# Autodesk Inventor assembly: fight_robot_fin1
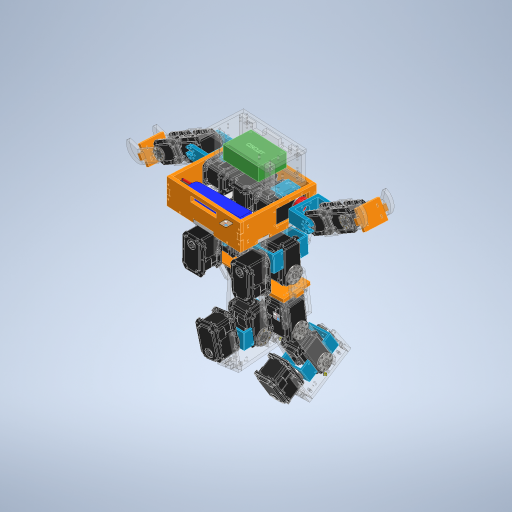
[picture p0: Inventor's stored thumbnail of the model, 512x512]
Saved by Autodesk Inventor 2024 (Build 280153000, 153)
## iProperties
Created: 2024-09-14
Part Number: fight_robot_fin1
Document SubType Name: Assembly
Designer: jmha0
Author: jmha0
## Documents named in this file (16)
- C:\Users\jmha0\OneDrive\바탕 화면\19th_intern_hjm_fight_robot\fight_robot_fin1.iam
- C:\Users\jmha0\OneDrive\바탕 화면\19th_intern_hjm_fight_robot\Lower_Body\waist\waist_fin1.iam
- C:\Users\jmha0\OneDrive\바탕 화면\19th_intern_hjm_fight_robot\Lower_Body\pelvis_w_motor\pelvis_w_motor_fin1.iam
- C:\Users\jmha0\OneDrive\바탕 화면\19th_intern_hjm_fight_robot\Lower_Body\pelvis_w_motor\pelvis_w_motor_fin1_opp.iam
- C:\Users\jmha0\OneDrive\바탕 화면\19th_intern_hjm_fight_robot\Lower_Body\knee_w_motor\knee_w_motor_fin1.iam
- C:\Users\jmha0\OneDrive\바탕 화면\19th_intern_hjm_fight_robot\Lower_Body\ankle_w_motor\ankle_w_motor_fin1.iam
- C:\Users\jmha0\OneDrive\바탕 화면\19th_intern_hjm_fight_robot\Lower_Body\ankle_w_motor\ankle_w_motor_fin1_opp.iam
- C:\Users\jmha0\OneDrive\바탕 화면\19th_intern_hjm_fight_robot\Lower_Body\feet\feet_fin1.iam
- C:\Users\jmha0\OneDrive\바탕 화면\19th_intern_hjm_fight_robot\Upper_Body\etc\long_horn1.ipt
- C:\Users\jmha0\OneDrive\바탕 화면\19th_intern_hjm_fight_robot\Upper_Body\Upper\upper_fin1.iam
- C:\Users\jmha0\OneDrive\바탕 화면\19th_intern_hjm_fight_robot\Upper_Body\arm\arm_fin1.iam
- C:\Users\jmha0\OneDrive\바탕 화면\19th_intern_hjm_fight_robot\Upper_Body\hand\hand_fin1.iam
- C:\Users\jmha0\OneDrive\바탕 화면\19th_intern_hjm_fight_robot\Upper_Body\hand\hand_fin1_opp.iam
- C:\Users\jmha0\OneDrive\바탕 화면\19th_intern_hjm_fight_robot\Upper_Body\head\head_fin1.iam
- C:\Users\jmha0\OneDrive\바탕 화면\19th_intern_hjm_fight_robot\battery\Enrichpower_2200mAh_11.1V_30C.ipt
- C:\Users\jmha0\OneDrive\바탕 화면\19th_intern_hjm_fight_robot\circuit\Circuit.ipt
## Components (20 placed, 15 different names)
1. waist_fin1:1 [sub-assembly] — 메이트:1, 메이트:2, 각도:1, 각도:2, 삽입:22, 삽입:23, 삽입:24, 삽입:26, 삽입:27
2. pelvis_w_motor_fin1:1 [sub-assembly] — 삽입:7, 삽입:8, 메이트:1, 각도:2
3. pelvis_w_motor_fin1_opp:1 [sub-assembly] — 삽입:9, 삽입:10, 메이트:2, 각도:1
4. knee_w_motor_fin1:1 [sub-assembly] — 삽입:7, 삽입:8, 삽입:14, 삽입:15
5. knee_w_motor_fin1:2 [sub-assembly] — 삽입:9, 삽입:10, 삽입:11, 삽입:12, 삽입:13
6. ankle_w_motor_fin1:1 [sub-assembly] — 삽입:11, 삽입:12, 삽입:13, 삽입:19, 삽입:20, 삽입:21
7. ankle_w_motor_fin1_opp:1 [sub-assembly] — 삽입:14, 삽입:15, 메이트:5
8. feet_fin1:1 [sub-assembly] — 메이트:5
9. feet_fin1:2 [sub-assembly] — 삽입:19, 삽입:20, 삽입:21
10. long_horn1:1 — 삽입:22, 삽입:23, 삽입:24, 삽입:25, 삽입:26, 삽입:27
11. upper_fin1:1 [sub-assembly] — 삽입:25, 삽입:28, 삽입:29, 삽입:30, 삽입:31, 삽입:32, 삽입:43, 삽입:44, 메이트:3
12. long_horn1:2 — 삽입:28, 삽입:29, 삽입:33, 삽입:34
13. long_horn1:3 — 삽입:30, 삽입:31, 삽입:32, 삽입:35, 삽입:36
14. arm_fin1:1 [sub-assembly] — 삽입:33, 삽입:34, 삽입:37, 삽입:38, 삽입:39
15. arm_fin1:2 [sub-assembly] — 삽입:35, 삽입:36, 삽입:40, 삽입:41, 삽입:42
16. hand_fin1:1 [sub-assembly] — 삽입:37, 삽입:38, 삽입:39
17. hand_fin1_opp:1 [sub-assembly] — 삽입:40, 삽입:41, 삽입:42
18. head_fin1:1 [sub-assembly] — 삽입:43, 삽입:44, 메이트:4
19. Enrichpower_2200mAh_11.1V_30C:1 — 메이트:3
20. Circuit:1 — 메이트:4
## Relationships (42: Insert 35, Mate 5, Angle 2)
- 삽입:7 [Insert]: pelvis_w_motor_fin1:1 ↔ knee_w_motor_fin1:1
- 삽입:8 [Insert]: pelvis_w_motor_fin1:1 ↔ knee_w_motor_fin1:1
- 삽입:9 [Insert]: pelvis_w_motor_fin1_opp:1 ↔ knee_w_motor_fin1:2
- 삽입:10 [Insert]: pelvis_w_motor_fin1_opp:1 ↔ knee_w_motor_fin1:2
- 삽입:11 [Insert]: knee_w_motor_fin1:2 ↔ ankle_w_motor_fin1:1
- 삽입:12 [Insert]: knee_w_motor_fin1:2 ↔ ankle_w_motor_fin1:1
- 삽입:13 [Insert]: knee_w_motor_fin1:2 ↔ ankle_w_motor_fin1:1
- 삽입:14 [Insert]: knee_w_motor_fin1:1 ↔ ankle_w_motor_fin1_opp:1
- 삽입:15 [Insert]: knee_w_motor_fin1:1 ↔ ankle_w_motor_fin1_opp:1
- 삽입:19 [Insert]: ankle_w_motor_fin1:1 ↔ feet_fin1:2
- 삽입:20 [Insert]: ankle_w_motor_fin1:1 ↔ feet_fin1:2
- 삽입:21 [Insert]: ankle_w_motor_fin1:1 ↔ feet_fin1:2
- 메이트:1 [Mate]: waist_fin1:1 ↔ pelvis_w_motor_fin1:1
- 메이트:2 [Mate]: waist_fin1:1 ↔ pelvis_w_motor_fin1_opp:1
- 각도:1 [Angle] (0 deg): waist_fin1:1 ↔ pelvis_w_motor_fin1_opp:1
- 각도:2 [Angle] (0 deg): waist_fin1:1 ↔ pelvis_w_motor_fin1:1
- 삽입:22 [Insert]: waist_fin1:1 ↔ long_horn1:1
- 삽입:23 [Insert]: waist_fin1:1 ↔ long_horn1:1
- 삽입:24 [Insert]: waist_fin1:1 ↔ long_horn1:1
- 삽입:25 [Insert]: long_horn1:1 ↔ upper_fin1:1
- 삽입:26 [Insert]: waist_fin1:1 ↔ long_horn1:1
- 삽입:27 [Insert]: waist_fin1:1 ↔ long_horn1:1
- 삽입:28 [Insert]: upper_fin1:1 ↔ long_horn1:2
- 삽입:29 [Insert]: upper_fin1:1 ↔ long_horn1:2
- 삽입:30 [Insert]: upper_fin1:1 ↔ long_horn1:3
- 삽입:31 [Insert]: upper_fin1:1 ↔ long_horn1:3
- 삽입:32 [Insert]: upper_fin1:1 ↔ long_horn1:3
- 삽입:33 [Insert]: long_horn1:2 ↔ arm_fin1:1
- 삽입:34 [Insert]: long_horn1:2 ↔ arm_fin1:1
- 삽입:35 [Insert]: long_horn1:3 ↔ arm_fin1:2
- 삽입:36 [Insert]: long_horn1:3 ↔ arm_fin1:2
- 삽입:37 [Insert]: arm_fin1:1 ↔ hand_fin1:1
- 삽입:38 [Insert]: arm_fin1:1 ↔ hand_fin1:1
- 삽입:39 [Insert]: arm_fin1:1 ↔ hand_fin1:1
- 삽입:40 [Insert]: arm_fin1:2 ↔ hand_fin1_opp:1
- 삽입:41 [Insert]: arm_fin1:2 ↔ hand_fin1_opp:1
- 삽입:42 [Insert]: arm_fin1:2 ↔ hand_fin1_opp:1
- 삽입:43 [Insert]: upper_fin1:1 ↔ head_fin1:1
- 삽입:44 [Insert]: upper_fin1:1 ↔ head_fin1:1
- 메이트:3 [Mate]: upper_fin1:1 ↔ Enrichpower_2200mAh_11.1V_30C:1
- 메이트:4 [Mate]: head_fin1:1 ↔ Circuit:1
- 메이트:5 [Mate]: ankle_w_motor_fin1_opp:1 ↔ feet_fin1:1
